# Autodesk Inventor assembly: ASDSAssembly
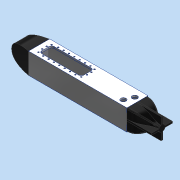
[picture p0: Inventor's stored thumbnail of the model, 180x180]
Saved by Autodesk Inventor 2018 (Build 220112000, 112)
## iProperties
Created: 2017-02-12
Part Number: ASDSAssembly
Document SubType Name: Assembly
Designer: techn
Author: techn
## Documents named in this file (7)
- D:\Projects\Submarine-project\CAD\ASDS\ASDSAssembly.iam
- D:\Projects\Submarine-project\CAD\ASDS\Fore.ipt
- D:\Projects\Submarine-project\CAD\ASDS\Aft.ipt
- D:\Projects\Submarine-project\CAD\ASDS\Hull_Alu.ipt
- D:\Projects\Submarine-project\CAD\ASDS\ForeAftMountPlate.ipt
- D:\Projects\Submarine-project\CAD\ASDS\TetherGuide.ipt
- D:\Projects\Submarine-project\CAD\common\ThreadedRod_Nuts_Bolts\Bolt_SocketHead_Hex_Thread_5_40_7_16length.ipt
## Components (8 placed, 6 different names)
1. Fore:1 — Mate:1, Mate:2, Mate:3, Mate:7, Mate:8, Mate:9
2. Hull_Alu:1 — Mate:1, Mate:2, Mate:3, Mate:4, Mate:5, Mate:6, Mate:13, Mate:14, Mate:15
3. Aft:1 — Mate:4, Mate:5, Mate:6, Mate:10, Mate:11, Mate:12
4. ForeAftMountPlate:1 — Mate:7, Mate:8, Mate:9
5. ForeAftMountPlate:2 — Mate:10, Mate:11, Mate:12
6. TetherGuide:1 — Mate:13, Mate:14, Mate:15, Mate:16, Mate:17, Mate:18, Angle:1, Mate:19, Angle:2
7. Bolt_SocketHead_Hex_Thread_5_40_7_16length:1 — Mate:16, Mate:18, Angle:1
8. Bolt_SocketHead_Hex_Thread_5_40_7_16length:2 — Mate:17, Mate:19, Angle:2
## Relationships (21: Mate 19, Angle 2)
- Mate:1: Fore:1 ↔ Hull_Alu:1
- Mate:2: Fore:1 ↔ Hull_Alu:1
- Mate:3: Fore:1 ↔ Hull_Alu:1
- Mate:4: Hull_Alu:1 ↔ Aft:1
- Mate:5: Hull_Alu:1 ↔ Aft:1
- Mate:6: Hull_Alu:1 ↔ Aft:1
- Mate:7: Fore:1 ↔ ForeAftMountPlate:1
- Mate:8: Fore:1 ↔ ForeAftMountPlate:1
- Mate:9: Fore:1 ↔ ForeAftMountPlate:1
- Mate:10: Aft:1 ↔ ForeAftMountPlate:2
- Mate:11: Aft:1 ↔ ForeAftMountPlate:2
- Mate:12: Aft:1 ↔ ForeAftMountPlate:2
- Mate:13: Hull_Alu:1 ↔ TetherGuide:1
- Mate:14: Hull_Alu:1 ↔ TetherGuide:1
- Mate:15: Hull_Alu:1 ↔ TetherGuide:1
- Mate:16: TetherGuide:1 ↔ Bolt_SocketHead_Hex_Thread_5_40_7_16length:1
- Mate:17: TetherGuide:1 ↔ Bolt_SocketHead_Hex_Thread_5_40_7_16length:2
- Mate:18: TetherGuide:1 ↔ Bolt_SocketHead_Hex_Thread_5_40_7_16length:1
- Angle:1 (0 deg): TetherGuide:1 ↔ Bolt_SocketHead_Hex_Thread_5_40_7_16length:1
- Mate:19: TetherGuide:1 ↔ Bolt_SocketHead_Hex_Thread_5_40_7_16length:2
- Angle:2 (0 deg): TetherGuide:1 ↔ Bolt_SocketHead_Hex_Thread_5_40_7_16length:2
